# Autodesk Inventor assembly: Extruder Side Panel Assembly
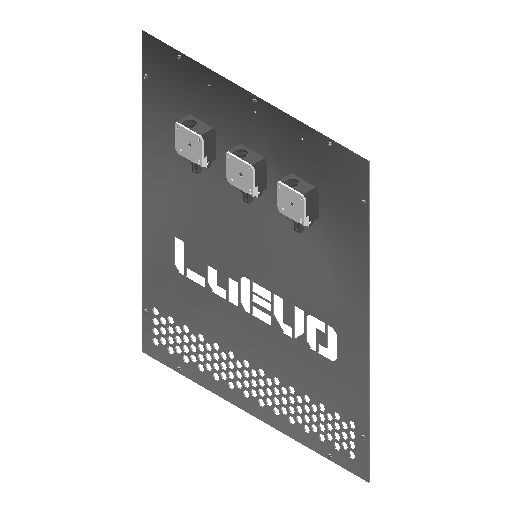
[picture p0: Inventor's stored thumbnail of the model, 512x512]
Saved by Autodesk Inventor 2023.2 (Build 272271000, 271)
## iProperties
Created: 2023-02-06
Part Number: Extruder Side Panel Assembly
Document SubType Name: Assembly
Designer: remop
Author: remop
## Documents named in this file (5)
- C:\Users\remop\OneDrive\Documents\Inventor\3D Printers\LuEVO\Mk5_FullKinematic\Extruder Side Panel Assembly.iam
- C:\Users\remop\OneDrive\Documents\Inventor\3D Printers\LuEVO\Mk5_FullKinematic\Extruder Side Panel.ipt
- C:\Users\remop\OneDrive\Documents\Inventor\3D Printers\LuEVO\Mk5_FullKinematic\Titan Extruder\e3d titan.iam
- C:\Users\remop\OneDrive\Documents\Inventor\3D Printers\LuEVO\Mk5_FullKinematic\Extruder Motor.ipt
- C:\Users\remop\OneDrive\Documents\Inventor\Content Center Files\R2023\en-US\AS 1420\AS 1420 - 1973 - M3 x 6.ipt
## Components (16 placed, 4 different names)
1. Extruder Side Panel:1 — Rotational:1, Rotational:2, Mate:1, Mate:2, Rigid:1, Rigid:2, Rigid:3, Rigid:4, Insert:1, Insert:14, Insert:15, Insert:16, Insert:17, Insert:18, Insert:19, Insert:20, Insert:21
2. e3d titan:1 [sub-assembly] — Rigid:1
3. e3d titan:2 [sub-assembly] — Rotational:1, Mate:1
4. e3d titan:3 [sub-assembly] — Rotational:2, Mate:2
5. Extruder Motor:1 — Rigid:2
6. Extruder Motor:2 — Rigid:3
7. Extruder Motor:3 — Rigid:4
8. AS 1420 - Metric M3 x 6:1 — Insert:1
9. AS 1420 - Metric M3 x 6:14 — Insert:14
10. AS 1420 - Metric M3 x 6:15 — Insert:15
11. AS 1420 - Metric M3 x 6:16 — Insert:16
12. AS 1420 - Metric M3 x 6:17 — Insert:17
13. AS 1420 - Metric M3 x 6:18 — Insert:18
14. AS 1420 - Metric M3 x 6:19 — Insert:19
15. AS 1420 - Metric M3 x 6:20 — Insert:20
16. AS 1420 - Metric M3 x 6:21 — Insert:21
## Relationships (17: Insert 9, WeldJoint 4, RevoluteJoint 2, Mate 2)
- Rotational:1 [RevoluteJoint]: Extruder Side Panel:1 ↔ e3d titan:2
- Rotational:2 [RevoluteJoint]: Extruder Side Panel:1 ↔ e3d titan:3
- Mate:1: Extruder Side Panel:1 ↔ e3d titan:2
- Mate:2: Extruder Side Panel:1 ↔ e3d titan:3
- Rigid:1 [WeldJoint]: Extruder Side Panel:1 ↔ e3d titan:1
- Rigid:2 [WeldJoint]: Extruder Side Panel:1 ↔ Extruder Motor:1
- Rigid:3 [WeldJoint]: Extruder Side Panel:1 ↔ Extruder Motor:2
- Rigid:4 [WeldJoint]: Extruder Side Panel:1 ↔ Extruder Motor:3
- Insert:1: Extruder Side Panel:1 ↔ AS 1420 - Metric M3 x 6:1
- Insert:14: Extruder Side Panel:1 ↔ AS 1420 - Metric M3 x 6:14
- Insert:15: Extruder Side Panel:1 ↔ AS 1420 - Metric M3 x 6:15
- Insert:16: Extruder Side Panel:1 ↔ AS 1420 - Metric M3 x 6:16
- Insert:17: Extruder Side Panel:1 ↔ AS 1420 - Metric M3 x 6:17
- Insert:18: Extruder Side Panel:1 ↔ AS 1420 - Metric M3 x 6:18
- Insert:19: Extruder Side Panel:1 ↔ AS 1420 - Metric M3 x 6:19
- Insert:20: Extruder Side Panel:1 ↔ AS 1420 - Metric M3 x 6:20
- Insert:21: Extruder Side Panel:1 ↔ AS 1420 - Metric M3 x 6:21
